# Autodesk Inventor assembly: Scanner-Assembly
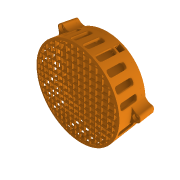
[picture p0: Inventor's stored thumbnail of the model, 180x180]
Saved by Autodesk Inventor 2020.3 (Build 243373000, 373)
## iProperties
Created: 2021-08-29
Part Number: Scanner-Assembly
Document SubType Name: Assembly
Designer: Yusuf
Mass: 67.0732 g
Surface Area: 694.358 cm^2
Volume: 67.0732 cm^3
Density: 1 g/cm^3
Author: Yusuf
## Documents named in this file (4)
- C:\Users\Yusuf\Desktop\BordaAcademy_BoxDesign\ESP32-Scanner\Scanner-Assembly.iam
- C:\Users\Yusuf\Desktop\BordaAcademy_BoxDesign\ESP32-Scanner\Scanner-BottomPart.ipt
- C:\Users\Yusuf\Desktop\BordaAcademy_BoxDesign\ESP32-Scanner\Scanner-TopPartV2.ipt
- C:\Users\Yusuf\Desktop\BordaAcademy_BoxDesign\ESP32-Scanner\Scanner-TopPartV2_MirrorV2.ipt
## Components (3 placed, 3 different names)
1. Scanner-BottomPart:1 — Mate:1, Mate:2, Mate:3, Mate:4, Mate:5, Mate:6, Mate:7
2. Scanner-TopPartV2:1 — Mate:4, Mate:5
3. Scanner-TopPartV2_MirrorV2:1 — Mate:6, Mate:7
## Relationships (7: Mate 7)
- Mate:1: Scanner-BottomPart:1
- Mate:2: Scanner-BottomPart:1
- Mate:3: Scanner-BottomPart:1
- Mate:4: Scanner-BottomPart:1 ↔ Scanner-TopPartV2:1
- Mate:5: Scanner-BottomPart:1 ↔ Scanner-TopPartV2:1
- Mate:6: Scanner-BottomPart:1 ↔ Scanner-TopPartV2_MirrorV2:1
- Mate:7: Scanner-BottomPart:1 ↔ Scanner-TopPartV2_MirrorV2:1
